# Autodesk Inventor assembly: shooting Mechanism
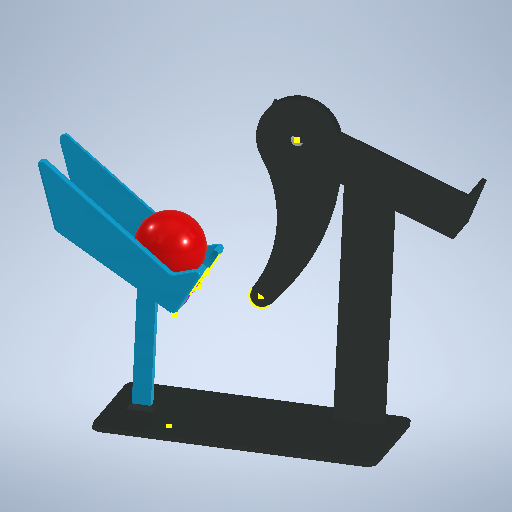
[picture p0: Inventor's stored thumbnail of the model, 512x512]
Saved by Autodesk Inventor 2025.4 (Build 294407000, 407)
## iProperties
Created: 2026-03-03
Part Number: shooting Mechanism
Document SubType Name: Assembly
Designer: youse
Author: youse
## Documents named in this file (4)
- D:\basics project\shooting Mechanism - Copy.iam
- D:\basics project\shooter.ipt
- D:\basics project\testing ball.ipt
- D:\basics project\shooting slider - Copy.ipt
## Components (3 placed, 3 different names)
1. shooter:1 — Mate:2, Mate:3
2. testing ball:1 — Tangent:1, Mate:1
3. shooting slider - Copy:1 — Tangent:1, Mate:1, Mate:2, Mate:3
## Relationships (4: Mate 3, Tangent 1)
- Tangent:1: testing ball:1 ↔ shooting slider - Copy:1
- Mate:1: testing ball:1 ↔ shooting slider - Copy:1
- Mate:2: shooter:1 ↔ shooting slider - Copy:1
- Mate:3: shooter:1 ↔ shooting slider - Copy:1
